# Autodesk Inventor assembly: lowerAssembly
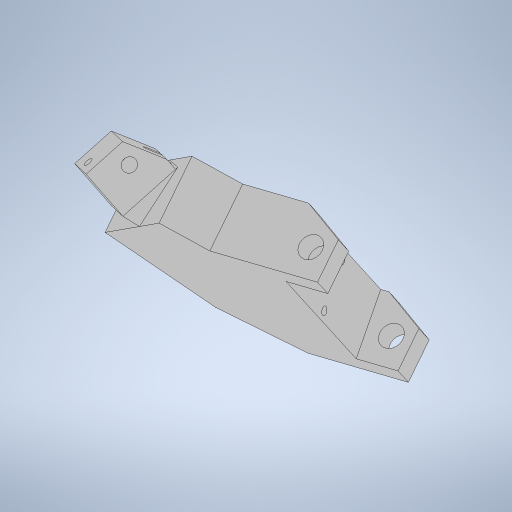
[picture p0: Inventor's stored thumbnail of the model, 512x512]
Saved by Autodesk Inventor 2024 (Build 280153000, 153)
## iProperties
Created: 2024-06-16
Part Number: lowerAssembly
Document SubType Name: Assembly
Designer: omiye
Author: omiye
## Documents named in this file (3)
- C:\Projects\roboticHand\fingerModels\fingerThumb\lowerAssembly.iam
- C:\Projects\roboticHand\fingerModels\normMale.ipt
- C:\Projects\roboticHand\fingerModels\fingerThumb\lower.ipt
## Components (2 placed, 2 different names)
1. lower:2 — Mate:12, Mate:13, Mate:14
2. normMale:1 — Mate:12, Mate:13, Mate:14
## Relationships (3: Mate 3)
- Mate:12: lower:2 ↔ normMale:1
- Mate:13: lower:2 ↔ normMale:1
- Mate:14: lower:2 ↔ normMale:1
